# Autodesk Inventor assembly: Main_assssembly
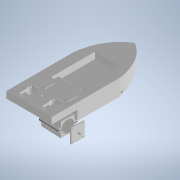
[picture p0: Inventor's stored thumbnail of the model, 180x180]
Saved by Autodesk Inventor 2020.1 (Build 241239000, 239)
## iProperties
Created: 2022-02-07
Part Number: Main_assssembly
Document SubType Name: Assembly
Designer: OEM
Author: OEM
## Documents named in this file (11)
- D:\Studia\Bobr\Repo\CAD\Main_assssembly.iam
- D:\Studia\Bobr\Repo\CAD\MainBody.ipt
- D:\Studia\Bobr\Repo\CAD\connector_sleeve.ipt
- D:\Studia\Bobr\Repo\CAD\engine_cup.ipt
- D:\Studia\Bobr\Repo\CAD\engine_lid.ipt
- D:\Studia\Bobr\Repo\CAD\engine_sleeve_up.ipt
- D:\Studia\Bobr\Repo\CAD\Bought_parts\Seal.ipt
- D:\Studia\Bobr\Repo\CAD\engine_sleeve_down.ipt
- D:\Studia\Bobr\Repo\CAD\Bought_parts\motor_subsitude.ipt
- D:\Studia\Bobr\Repo\CAD\engine_gear_connector.ipt
- D:\Studia\Bobr\Repo\CAD\back_axis.ipt
## Components (11 placed, 10 different names)
1. MainBody:2 — Rotational:1, Mate:6
2. connector_sleeve:1 — Rotational:1, Mate:5
3. engine_cup:1 — Rigid:5, Mate:7, Mate:8, Mate:9
4. engine_lid:1 — Rotational:2, Mate:19, Mate:20, Mate:21
5. engine_sleeve_up:1 — Mate:5, Mate:6, Rigid:5, Mate:12, Mate:13, Rigid:6, Rigid:7, Mate:19, Mate:20
6. Seal:1 — Mate:16, Mate:17, Rigid:7
7. Seal:2 — Mate:12, Mate:13, Rigid:6, Mate:14, Mate:15
8. engine_sleeve_down:1 — Mate:14, Mate:15, Mate:16, Mate:17, Mate:21
9. motor_subsitude:1 — Mate:7, Mate:8, Mate:9, Mate:10, Mate:11
10. engine_gear_connector:2 — Mate:10, Mate:11
11. back_axis:1 — Rotational:2
## Relationships (21: Mate 16, WeldJoint 3, RevoluteJoint 2)
- Rotational:1 [RevoluteJoint]: MainBody:2 ↔ connector_sleeve:1
- Mate:5: connector_sleeve:1 ↔ engine_sleeve_up:1
- Mate:6: MainBody:2 ↔ engine_sleeve_up:1
- Rigid:5 [WeldJoint]: engine_cup:1 ↔ engine_sleeve_up:1
- Mate:7: engine_cup:1 ↔ motor_subsitude:1
- Mate:8: engine_cup:1 ↔ motor_subsitude:1
- Mate:9: engine_cup:1 ↔ motor_subsitude:1
- Mate:10: motor_subsitude:1 ↔ engine_gear_connector:2
- Mate:11: motor_subsitude:1 ↔ engine_gear_connector:2
- Rotational:2 [RevoluteJoint]: engine_lid:1 ↔ back_axis:1
- Mate:12: engine_sleeve_up:1 ↔ Seal:2
- Mate:13: engine_sleeve_up:1 ↔ Seal:2
- Rigid:6 [WeldJoint]: engine_sleeve_up:1 ↔ Seal:2
- Mate:14: Seal:2 ↔ engine_sleeve_down:1
- Mate:15: Seal:2 ↔ engine_sleeve_down:1
- Mate:16: Seal:1 ↔ engine_sleeve_down:1
- Mate:17: Seal:1 ↔ engine_sleeve_down:1
- Rigid:7 [WeldJoint]: engine_sleeve_up:1 ↔ Seal:1
- Mate:19: engine_lid:1 ↔ engine_sleeve_up:1
- Mate:20: engine_lid:1 ↔ engine_sleeve_up:1
- Mate:21: engine_lid:1 ↔ engine_sleeve_down:1
